# Autodesk Inventor assembly: 試作1
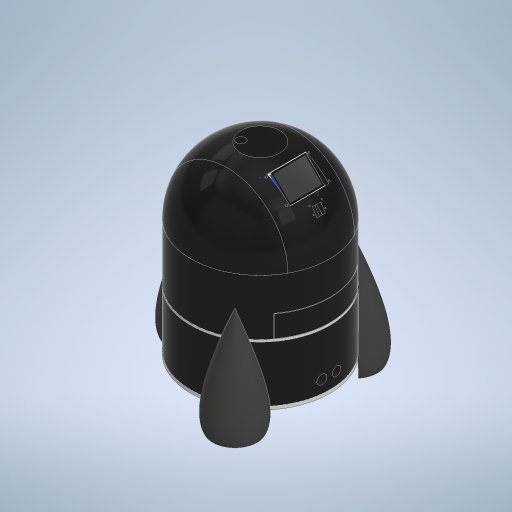
[picture p0: Inventor's stored thumbnail of the model, 512x512]
Saved by Autodesk Inventor 2023 (Build 270158000, 158)
## iProperties
Created: 2022-11-18
Part Number: 試作1
Document SubType Name: Assembly
Designer: 野口　裕太
Author: 野口　裕太
## Documents named in this file (9)
- E:\ロボ創\試作1.iam
- E:\ロボ創\底板 (2).ipt
- E:\ロボ創\newbody6.ipt
- E:\ロボ創\newbody5.ipt
- E:\ロボ創\newleg.ipt
- E:\ロボ創\newhead.ipt
- E:\ロボ創\Part11.ipt
- C:\Users\yuta\Downloads\2-8in-lcd-module-1.snapshot.11\2.8 TFT Module.iam
- E:\ロボ創\お盆試作2.iam
## Components (12 placed, 8 different names)
1. 底板 (2):1 — メイト:1, メイト:2, メイト:3, メイト:4, メイト:5, メイト:6, メイト:8, メイト:9, メイト:10
2. newbody6:1 — メイト:1, メイト:2, メイト:3, メイト:7, メイト:12, メイト:13
3. newbody5:1 — メイト:8, メイト:9, メイト:10, メイト:11
4. newbody5:2 — メイト:4, メイト:5, メイト:6, メイト:7, メイト:14, メイト:15, メイト:16, メイト:28, メイト:29
5. newleg:1 — メイト:13, メイト:14
6. newleg:2 — メイト:11, メイト:12
7. newleg:3 — メイト:15, メイト:16
8. newhead:1 — メイト:21, メイト:25, メイト:30, メイト:31, メイト:32, メイト:33, メイト:34, メイト:35
9. Part11:1 — メイト:21, メイト:31
10. Part11:2 — メイト:25, メイト:30
11. お盆試作2:1 [sub-assembly] — メイト:28, メイト:29, メイト:32, メイト:33
12. 2.8 TFT Module:1 [sub-assembly] — メイト:34, メイト:35
## Relationships (26: Mate 26)
- メイト:1 [Mate]: 底板 (2):1 ↔ newbody6:1
- メイト:2 [Mate]: 底板 (2):1 ↔ newbody6:1
- メイト:3 [Mate]: 底板 (2):1 ↔ newbody6:1
- メイト:4 [Mate]: 底板 (2):1 ↔ newbody5:2
- メイト:5 [Mate]: 底板 (2):1 ↔ newbody5:2
- メイト:6 [Mate]: 底板 (2):1 ↔ newbody5:2
- メイト:7 [Mate]: newbody6:1 ↔ newbody5:2
- メイト:8 [Mate]: 底板 (2):1 ↔ newbody5:1
- メイト:9 [Mate]: 底板 (2):1 ↔ newbody5:1
- メイト:10 [Mate]: 底板 (2):1 ↔ newbody5:1
- メイト:11 [Mate]: newbody5:1 ↔ newleg:2
- メイト:12 [Mate]: newbody6:1 ↔ newleg:2
- メイト:13 [Mate]: newbody6:1 ↔ newleg:1
- メイト:14 [Mate]: newbody5:2 ↔ newleg:1
- メイト:15 [Mate]: newbody5:2 ↔ newleg:3
- メイト:16 [Mate]: newbody5:2 ↔ newleg:3
- メイト:21 [Mate]: newhead:1 ↔ Part11:1
- メイト:25 [Mate]: newhead:1 ↔ Part11:2
- メイト:28 [Mate]: newbody5:2 ↔ お盆試作2:1
- メイト:29 [Mate]: newbody5:2 ↔ お盆試作2:1
- メイト:30 [Mate]: newhead:1 ↔ Part11:2
- メイト:31 [Mate]: newhead:1 ↔ Part11:1
- メイト:32 [Mate]: newhead:1 ↔ お盆試作2:1
- メイト:33 [Mate]: newhead:1 ↔ お盆試作2:1
- メイト:34 [Mate]: newhead:1 ↔ 2.8 TFT Module:1
- メイト:35 [Mate]: newhead:1 ↔ 2.8 TFT Module:1
